# Autodesk Inventor assembly: Ensamblaje1
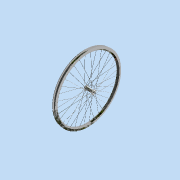
[picture p0: Inventor's stored thumbnail of the model, 180x180]
Saved by Autodesk Inventor 2017 (Build 210142000, 142)
## iProperties
Part Number: Ensamblaje1
Material: Genérico
Document SubType Name: Assembly
Designer: Miguel A.
Author: Miguel A.
## Documents named in this file (8)
- \\192.168.1.220\Proyectos\rueda de moto\Ensamblaje1.iam
- \\192.168.1.220\Proyectos\rueda de moto\buje.ipt
- \\192.168.1.220\Proyectos\rueda de moto\eje roscado.ipt
- \\192.168.1.220\Proyectos\rueda de moto\bola.ipt
- \\192.168.1.220\Proyectos\rueda de moto\tuerca bola.ipt
- \\192.168.1.220\Proyectos\rueda de moto\llanta.ipt
- \\192.168.1.220\Proyectos\rueda de moto\tornillo.ipt
- \\192.168.1.220\Proyectos\rueda de moto\radio.ipt
## Components (93 placed, 7 different names)
1. eje roscado:1 — Coincidencia:1, Coincidencia:2, Coincidencia:3, Coincidencia:4, Nivelación:1, Coincidencia:5, Coincidencia:6, Coincidencia:7
2. buje:1 — Coincidencia:4, Nivelación:1, Tangente:4, Tangente:6, Coincidencia:8, Coincidencia:9, Coincidencia:46, Coincidencia:48, Coincidencia:50, Coincidencia:52, Coincidencia:54, Coincidencia:56, Coincidencia:58, Coincidencia:60, Coincidencia:62, Coincidencia:64, Coincidencia:66, Coincidencia:68, Coincidencia:70, Coincidencia:72, Coincidencia:74, Coincidencia:76, Coincidencia:78, Coincidencia:80, Coincidencia:82, Coincidencia:99, Coincidencia:100, Coincidencia:101, Coincidencia:102, Coincidencia:103, Coincidencia:104, Coincidencia:105, Coincidencia:106, Coincidencia:108, Coincidencia:110, Coincidencia:112, Coincidencia:114, Coincidencia:116, Coincidencia:118, Coincidencia:120, Coincidencia:122, Coincidencia:124
3. tuerca bola:1 — Coincidencia:5, Tangente:5
4. tuerca bola:2 — Coincidencia:7, Tangente:7
5. llanta:1 — Coincidencia:8, Coincidencia:9, Coincidencia:10, Coincidencia:11, Coincidencia:12, Coincidencia:13, Coincidencia:14, Coincidencia:15, Coincidencia:16, Coincidencia:17, Coincidencia:18, Coincidencia:19, Coincidencia:20, Coincidencia:21, Coincidencia:22, Coincidencia:23, Coincidencia:24, Coincidencia:25, Coincidencia:26, Coincidencia:27, Coincidencia:28, Coincidencia:29, Coincidencia:30, Coincidencia:31, Coincidencia:32, Coincidencia:33, Coincidencia:34, Coincidencia:35, Coincidencia:36, Coincidencia:37, Coincidencia:38, Coincidencia:39, Coincidencia:40, Coincidencia:41, Coincidencia:42, Coincidencia:43, Coincidencia:44, Coincidencia:45
6. tornillo:1 — Coincidencia:10, Coincidencia:123
7. tornillo:7 — Coincidencia:12, Coincidencia:83
8. tornillo:15 — Coincidencia:23, Coincidencia:77
9. tornillo:16 — Coincidencia:20, Coincidencia:87
10. tornillo:17 — Coincidencia:22, Coincidencia:117
11. tornillo:18 — Coincidencia:13, Coincidencia:49
12. tornillo:19 — Coincidencia:14, Coincidencia:121
13. tornillo:20 — Coincidencia:16, Coincidencia:85
14. tornillo:21 — Coincidencia:17, Coincidencia:47, Nivelación:2
15. tornillo:22 — Coincidencia:21, Coincidencia:63
16. tornillo:23 — Coincidencia:18, Coincidencia:119
17. tornillo:24 — Coincidencia:19, Coincidencia:75
18. tornillo:36 — Coincidencia:15, Coincidencia:73
19. tornillo:37 — Coincidencia:11, Coincidencia:71
20. tornillo:38 — Coincidencia:24, Coincidencia:89
21. tornillo:39 — Coincidencia:25, Coincidencia:61
22. tornillo:40 — Coincidencia:26, Coincidencia:115
23. tornillo:41 — Coincidencia:27, Coincidencia:79
24. tornillo:42 — Coincidencia:28, Coincidencia:91
25. tornillo:43 — Coincidencia:29, Coincidencia:59
26. tornillo:44 — Coincidencia:30, Coincidencia:113
27. tornillo:45 — Coincidencia:31, Coincidencia:81
28. tornillo:46 — Coincidencia:32, Coincidencia:93
29. tornillo:47 — Coincidencia:33, Coincidencia:57
30. tornillo:48 — Coincidencia:34, Coincidencia:111
31. tornillo:49 — Coincidencia:35, Coincidencia:65
32. tornillo:50 — Coincidencia:36, Coincidencia:95
33. tornillo:51 — Coincidencia:37, Coincidencia:55
34. tornillo:52 — Coincidencia:38, Coincidencia:109
35. tornillo:53 — Coincidencia:39, Coincidencia:67
36. tornillo:54 — Coincidencia:40, Coincidencia:97
37. tornillo:55 — Coincidencia:41, Coincidencia:53
38. tornillo:56 — Coincidencia:42, Coincidencia:125
39. tornillo:57 — Coincidencia:43, Coincidencia:69
40. tornillo:58 — Coincidencia:45, Coincidencia:51
41. tornillo:59 — Coincidencia:44, Coincidencia:107
42. radio:1 — Coincidencia:46, Coincidencia:47, Nivelación:2
43. radio:2 — Coincidencia:48, Coincidencia:49
44. radio:3 — Coincidencia:50, Coincidencia:51
45. radio:4 — Coincidencia:52, Coincidencia:53
46. radio:5 — Coincidencia:54, Coincidencia:55
47. radio:6 — Coincidencia:56, Coincidencia:57
48. radio:7 — Coincidencia:58, Coincidencia:59
49. radio:8 — Coincidencia:60, Coincidencia:61
50. radio:9 — Coincidencia:62, Coincidencia:63
51. radio:10 — Coincidencia:64, Coincidencia:65
52. radio:11 — Coincidencia:66, Coincidencia:67
53. radio:12 — Coincidencia:68, Coincidencia:69
54. radio:13 — Coincidencia:70, Coincidencia:71
55. radio:14 — Coincidencia:72, Coincidencia:73
56. radio:15 — Coincidencia:74, Coincidencia:75
57. radio:16 — Coincidencia:76, Coincidencia:77
58. radio:17 — Coincidencia:78, Coincidencia:79
59. radio:18 — Coincidencia:80, Coincidencia:81
60. radio:19 — Coincidencia:82, Coincidencia:83
61. radio:20 — Coincidencia:85, Coincidencia:99
62. radio:21 — Coincidencia:87, Coincidencia:100
63. radio:22 — Coincidencia:89, Coincidencia:101
64. radio:23 — Coincidencia:91, Coincidencia:102
65. radio:24 — Coincidencia:93, Coincidencia:103
66. radio:25 — Coincidencia:95, Coincidencia:104
67. radio:26 — Coincidencia:97, Coincidencia:105
68. radio:27 — Coincidencia:106, Coincidencia:107
69. radio:28 — Coincidencia:108, Coincidencia:109
70. radio:29 — Coincidencia:110, Coincidencia:111
71. radio:30 — Coincidencia:112, Coincidencia:113
72. radio:31 — Coincidencia:114, Coincidencia:115
73. radio:32 — Coincidencia:116, Coincidencia:117
74. radio:33 — Coincidencia:118, Coincidencia:119
75. radio:34 — Coincidencia:120, Coincidencia:121
76. radio:35 — Coincidencia:122, Coincidencia:123
77. radio:36 — Coincidencia:124, Coincidencia:125
78. bola:14 — Tangente:4, Tangente:5
79. bola:15
80. bola:16
81. bola:17
82. bola:18
83. bola:19
84. bola:20
85. bola:21
86. bola:22 — Tangente:6, Tangente:7
87. bola:23
88. bola:24
89. bola:25
90. bola:26
91. bola:27
92. bola:28
93. bola:29
## Component patterns: (8 elements, first: bola:14), (8 elements, first: bola:22)
## Relationships (123: Mate 117, Tangent 4, Flush 2)
- Coincidencia:1 [Mate]: eje roscado:1
- Coincidencia:2 [Mate]: eje roscado:1
- Coincidencia:3 [Mate]: eje roscado:1
- Coincidencia:4 [Mate]: eje roscado:1 ↔ buje:1
- Nivelación:1 [Flush] (21 mm): eje roscado:1 ↔ buje:1
- Tangente:4: buje:1 ↔ bola:14
- Coincidencia:5 [Mate]: eje roscado:1 ↔ tuerca bola:1
- Tangente:5: tuerca bola:1 ↔ bola:14
- Coincidencia:6 [Mate]: eje roscado:1
- Tangente:6: buje:1 ↔ bola:22
- Coincidencia:7 [Mate]: eje roscado:1 ↔ tuerca bola:2
- Tangente:7: tuerca bola:2 ↔ bola:22
- Coincidencia:8 [Mate]: buje:1 ↔ llanta:1
- Coincidencia:9 [Mate]: buje:1 ↔ llanta:1
- Coincidencia:10 [Mate]: llanta:1 ↔ tornillo:1
- Coincidencia:11 [Mate]: llanta:1 ↔ tornillo:37
- Coincidencia:12 [Mate]: llanta:1 ↔ tornillo:7
- Coincidencia:13 [Mate]: llanta:1 ↔ tornillo:18
- Coincidencia:14 [Mate]: llanta:1 ↔ tornillo:19
- Coincidencia:15 [Mate]: llanta:1 ↔ tornillo:36
- Coincidencia:16 [Mate]: llanta:1 ↔ tornillo:20
- Coincidencia:17 [Mate]: llanta:1 ↔ tornillo:21
- Coincidencia:18 [Mate]: llanta:1 ↔ tornillo:23
- Coincidencia:19 [Mate]: llanta:1 ↔ tornillo:24
- Coincidencia:20 [Mate]: llanta:1 ↔ tornillo:16
- Coincidencia:21 [Mate]: llanta:1 ↔ tornillo:22
- Coincidencia:22 [Mate]: llanta:1 ↔ tornillo:17
- Coincidencia:23 [Mate]: llanta:1 ↔ tornillo:15
- Coincidencia:24 [Mate]: llanta:1 ↔ tornillo:38
- Coincidencia:25 [Mate]: llanta:1 ↔ tornillo:39
- Coincidencia:26 [Mate]: llanta:1 ↔ tornillo:40
- Coincidencia:27 [Mate]: llanta:1 ↔ tornillo:41
- Coincidencia:28 [Mate]: llanta:1 ↔ tornillo:42
- Coincidencia:29 [Mate]: llanta:1 ↔ tornillo:43
- Coincidencia:30 [Mate]: llanta:1 ↔ tornillo:44
- Coincidencia:31 [Mate]: llanta:1 ↔ tornillo:45
- Coincidencia:32 [Mate]: llanta:1 ↔ tornillo:46
- Coincidencia:33 [Mate]: llanta:1 ↔ tornillo:47
- Coincidencia:34 [Mate]: llanta:1 ↔ tornillo:48
- Coincidencia:35 [Mate]: llanta:1 ↔ tornillo:49
- Coincidencia:36 [Mate]: llanta:1 ↔ tornillo:50
- Coincidencia:37 [Mate]: llanta:1 ↔ tornillo:51
- Coincidencia:38 [Mate]: llanta:1 ↔ tornillo:52
- Coincidencia:39 [Mate]: llanta:1 ↔ tornillo:53
- Coincidencia:40 [Mate]: llanta:1 ↔ tornillo:54
- Coincidencia:41 [Mate]: llanta:1 ↔ tornillo:55
- Coincidencia:42 [Mate]: llanta:1 ↔ tornillo:56
- Coincidencia:43 [Mate]: llanta:1 ↔ tornillo:57
- Coincidencia:44 [Mate]: llanta:1 ↔ tornillo:59
- Coincidencia:45 [Mate]: llanta:1 ↔ tornillo:58
- Coincidencia:46 [Mate]: buje:1 ↔ radio:1
- Coincidencia:47 [Mate]: tornillo:21 ↔ radio:1
- Nivelación:2 [Flush]: tornillo:21 ↔ radio:1
- Coincidencia:48 [Mate]: buje:1 ↔ radio:2
- Coincidencia:49 [Mate]: tornillo:18 ↔ radio:2
- Coincidencia:50 [Mate]: buje:1 ↔ radio:3
- Coincidencia:51 [Mate]: tornillo:58 ↔ radio:3
- Coincidencia:52 [Mate]: buje:1 ↔ radio:4
- Coincidencia:53 [Mate]: tornillo:55 ↔ radio:4
- Coincidencia:54 [Mate]: buje:1 ↔ radio:5
- Coincidencia:55 [Mate]: tornillo:51 ↔ radio:5
- Coincidencia:56 [Mate]: buje:1 ↔ radio:6
- Coincidencia:57 [Mate]: tornillo:47 ↔ radio:6
- Coincidencia:58 [Mate]: buje:1 ↔ radio:7
- Coincidencia:59 [Mate]: tornillo:43 ↔ radio:7
- Coincidencia:60 [Mate]: buje:1 ↔ radio:8
- Coincidencia:61 [Mate]: tornillo:39 ↔ radio:8
- Coincidencia:62 [Mate]: buje:1 ↔ radio:9
- Coincidencia:63 [Mate]: tornillo:22 ↔ radio:9
- Coincidencia:64 [Mate]: buje:1 ↔ radio:10
- Coincidencia:65 [Mate]: tornillo:49 ↔ radio:10
- Coincidencia:66 [Mate]: buje:1 ↔ radio:11
- Coincidencia:67 [Mate]: tornillo:53 ↔ radio:11
- Coincidencia:68 [Mate]: buje:1 ↔ radio:12
- Coincidencia:69 [Mate]: tornillo:57 ↔ radio:12
- Coincidencia:70 [Mate]: buje:1 ↔ radio:13
- Coincidencia:71 [Mate]: tornillo:37 ↔ radio:13
- Coincidencia:72 [Mate]: buje:1 ↔ radio:14
- Coincidencia:73 [Mate]: tornillo:36 ↔ radio:14
- Coincidencia:74 [Mate]: buje:1 ↔ radio:15
- Coincidencia:75 [Mate]: tornillo:24 ↔ radio:15
- Coincidencia:76 [Mate]: buje:1 ↔ radio:16
- Coincidencia:77 [Mate]: tornillo:15 ↔ radio:16
- Coincidencia:78 [Mate]: buje:1 ↔ radio:17
- Coincidencia:79 [Mate]: tornillo:41 ↔ radio:17
- Coincidencia:80 [Mate]: buje:1 ↔ radio:18
- Coincidencia:81 [Mate]: tornillo:45 ↔ radio:18
- Coincidencia:82 [Mate]: buje:1 ↔ radio:19
- Coincidencia:83 [Mate]: tornillo:7 ↔ radio:19
- Coincidencia:85 [Mate]: tornillo:20 ↔ radio:20
- Coincidencia:87 [Mate]: tornillo:16 ↔ radio:21
- Coincidencia:89 [Mate]: tornillo:38 ↔ radio:22
- Coincidencia:91 [Mate]: tornillo:42 ↔ radio:23
- Coincidencia:93 [Mate]: tornillo:46 ↔ radio:24
- Coincidencia:95 [Mate]: tornillo:50 ↔ radio:25
- Coincidencia:97 [Mate]: tornillo:54 ↔ radio:26
- Coincidencia:99 [Mate]: buje:1 ↔ radio:20
- Coincidencia:100 [Mate]: buje:1 ↔ radio:21
- Coincidencia:101 [Mate]: buje:1 ↔ radio:22
- Coincidencia:102 [Mate]: buje:1 ↔ radio:23
- Coincidencia:103 [Mate]: buje:1 ↔ radio:24
- Coincidencia:104 [Mate]: buje:1 ↔ radio:25
- Coincidencia:105 [Mate]: buje:1 ↔ radio:26
- Coincidencia:106 [Mate]: buje:1 ↔ radio:27
- Coincidencia:107 [Mate]: tornillo:59 ↔ radio:27
- Coincidencia:108 [Mate]: buje:1 ↔ radio:28
- Coincidencia:109 [Mate]: tornillo:52 ↔ radio:28
- Coincidencia:110 [Mate]: buje:1 ↔ radio:29
- Coincidencia:111 [Mate]: tornillo:48 ↔ radio:29
- Coincidencia:112 [Mate]: buje:1 ↔ radio:30
- Coincidencia:113 [Mate]: tornillo:44 ↔ radio:30
- Coincidencia:114 [Mate]: buje:1 ↔ radio:31
- Coincidencia:115 [Mate]: tornillo:40 ↔ radio:31
- Coincidencia:116 [Mate]: buje:1 ↔ radio:32
- Coincidencia:117 [Mate]: tornillo:17 ↔ radio:32
- Coincidencia:118 [Mate]: buje:1 ↔ radio:33
- Coincidencia:119 [Mate]: tornillo:23 ↔ radio:33
- Coincidencia:120 [Mate]: buje:1 ↔ radio:34
- Coincidencia:121 [Mate]: tornillo:19 ↔ radio:34
- Coincidencia:122 [Mate]: buje:1 ↔ radio:35
- Coincidencia:123 [Mate]: tornillo:1 ↔ radio:35
- Coincidencia:124 [Mate]: buje:1 ↔ radio:36
- Coincidencia:125 [Mate]: tornillo:56 ↔ radio:36
